# Autodesk Inventor assembly: solar charger
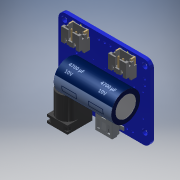
[picture p0: Inventor's stored thumbnail of the model, 180x180]
Saved by Autodesk Inventor 2019 (Build 230136000, 136)
## iProperties
Created: 2020-03-05
Part Number: solar charger
Document SubType Name: Assembly
Designer: ntb11189
Author: ntb11189
## Documents named in this file (6)
- N:\Sandpit\Callum Brooksby\Main Enclosure\Solar charger\solar charger.iam
- N:\Sandpit\Zack North\Group Project CAD\solar charger board.ipt
- C:\Users\ntb11189\Downloads\adafruit-jst-ph-2-pin-smt-right-angle-breakout-board-1.snapshot.1 (1)\S2B-PH-SM4-TB.ipt
- C:\Users\ntb11189\Downloads\mini-smd-usb-connector-female-1.snapshot.1\Mini USB.ipt
- C:\Users\ntb11189\Downloads\ninigi-pc-gk2-1-dc-1.snapshot.1\PC-GK2.1--3DModel-STEP-56544.ipt
- N:\Sandpit\Zack North\Group Project CAD\capacitor.ipt
## Components (6 placed, 5 different names)
1. Adafruit MCP73871 Solar Charger v4.brd_Outline:1 — Flush:1, Flush:2, Mate:4, Mate:5, Flush:3, Flush:4, Mate:6, Flush:5, Flush:6, Mate:7, Flush:7, Flush:8, Flush:9, Tangent:1, Mate:8
2. S2B-PH-SM4-TB:1 — Flush:1, Mate:4, Flush:4
3. S2B-PH-SM4-TB:2 — Flush:2, Mate:5, Flush:3
4. Mini USB:1 — Mate:6, Flush:5, Flush:6
5. PC-GK2.1--3DModel-STEP-56544:1 — Mate:7, Flush:7, Flush:8
6. capacitor:2 — Flush:9, Tangent:1, Mate:8
## Relationships (15: Flush 9, Mate 5, Tangent 1)
- Flush:1 (1 mm): Adafruit MCP73871 Solar Charger v4.brd_Outline:1 ↔ S2B-PH-SM4-TB:1
- Flush:2 (-1 mm): Adafruit MCP73871 Solar Charger v4.brd_Outline:1 ↔ S2B-PH-SM4-TB:2
- Mate:4: Adafruit MCP73871 Solar Charger v4.brd_Outline:1 ↔ S2B-PH-SM4-TB:1
- Mate:5: Adafruit MCP73871 Solar Charger v4.brd_Outline:1 ↔ S2B-PH-SM4-TB:2
- Flush:3 (6 mm): Adafruit MCP73871 Solar Charger v4.brd_Outline:1 ↔ S2B-PH-SM4-TB:2
- Flush:4 (6 mm): Adafruit MCP73871 Solar Charger v4.brd_Outline:1 ↔ S2B-PH-SM4-TB:1
- Mate:6: Adafruit MCP73871 Solar Charger v4.brd_Outline:1 ↔ Mini USB:1
- Flush:5 (-1 mm): Adafruit MCP73871 Solar Charger v4.brd_Outline:1 ↔ Mini USB:1
- Flush:6 (13 mm): Adafruit MCP73871 Solar Charger v4.brd_Outline:1 ↔ Mini USB:1
- Mate:7: Adafruit MCP73871 Solar Charger v4.brd_Outline:1 ↔ PC-GK2.1--3DModel-STEP-56544:1
- Flush:7 (-2 mm): Adafruit MCP73871 Solar Charger v4.brd_Outline:1 ↔ PC-GK2.1--3DModel-STEP-56544:1
- Flush:8 (-6 mm): Adafruit MCP73871 Solar Charger v4.brd_Outline:1 ↔ PC-GK2.1--3DModel-STEP-56544:1
- Flush:9 (3 mm): Adafruit MCP73871 Solar Charger v4.brd_Outline:1 ↔ capacitor:2
- Tangent:1 (-25 mm): Adafruit MCP73871 Solar Charger v4.brd_Outline:1 ↔ capacitor:2
- Mate:8 (8 mm): Adafruit MCP73871 Solar Charger v4.brd_Outline:1 ↔ capacitor:2
